# Autodesk Inventor assembly: EnsambleMarcador
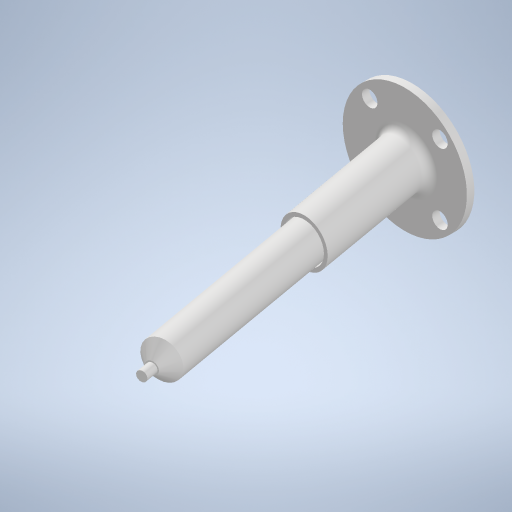
[picture p0: Inventor's stored thumbnail of the model, 512x512]
Saved by Autodesk Inventor 2023 (Build 270158000, 158)
## iProperties
Created: 2023-09-04
Part Number: EnsambleMarcador
Document SubType Name: Assembly
Designer: felip
Author: felip
## Documents named in this file (3)
- D:\UNAL\Robot\Labs\Lab1\CAD\EnsambleMarcador.iam
- D:\UNAL\Robot\Labs\Lab1\CAD\Marcador.ipt
- D:\UNAL\Robot\Labs\Lab1\CAD\SoporteMarcador.ipt
## Components (2 placed, 2 different names)
1. Marcador:1 — Mate:2
2. SoporteMarcador:1 — Mate:1, Mate:2
## Relationships (2: Mate 2)
- Mate:1: SoporteMarcador:1
- Mate:2: Marcador:1 ↔ SoporteMarcador:1
